# Autodesk Inventor assembly: Assembled_Olfactometer
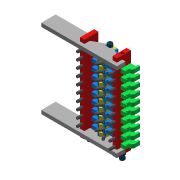
[picture p0: Inventor's stored thumbnail of the model, 180x180]
Saved by Autodesk Inventor 2016 (Build 200138000, 138)
## iProperties
Created: 2018-02-11
Part Number: Assembled_Olfactometer
Document SubType Name: Assembly
Designer: reinert
Author: reinert
## Documents named in this file (8)
- D:\PHD KUNER\Behaviour Setup\KunerOlfactometer_9Valves\Assembled_Olfactometer.iam
- D:\PHD KUNER\Behaviour Setup\KunerOlfactometer_9Valves\Olfactometer_Holder.ipt
- D:\PHD KUNER\Behaviour Setup\KunerOlfactometer_9Valves\OuterOlfactometerChannel.ipt
- D:\PHD KUNER\Behaviour Setup\KunerOlfactometer_9Valves\CentralManifold.ipt
- D:\PHD KUNER\Behaviour Setup\KunerOlfactometer_9Valves\Valve_Outside.ipt
- D:\PHD KUNER\Behaviour Setup\KunerOlfactometer_9Valves\Valve_Inside.ipt
- D:\PHD KUNER\Behaviour Setup\KunerOlfactometer_9Valves\KQ2S23_M5N_N.ipt
- D:\PHD KUNER\Behaviour Setup\KunerOlfactometer_9Valves\2027 CK-1_8-PK-4.ipt
## Components (89 placed, 7 different names)
1. Olfactometer_Holder:1 — Flush:1, Flush:2, Flush:3, Mate:1, Mate:3, Mate:4, Flush:5, Flush:6, Mate:5, Flush:9, Mate:6
2. Olfactometer_Holder:2 — Flush:1, Flush:2, Flush:3
3. OuterOlfactometerChannel:1 — Mate:1, Flush:9, Mate:6, Insert:1, Insert:2, Mate:8, Insert:11, Mate:14, Insert:16
4. OuterOlfactometerChannel:2 — Mate:3, Mate:4, Flush:5, Flush:8, Insert:3, Insert:4, Mate:7, Insert:9, Mate:13, Insert:15
5. CentralManifold:1 — Flush:6, Flush:8, Mate:5, Insert:5, Insert:6, Insert:7, Insert:8, Mate:9, Insert:10, Mate:10, Insert:12, Mate:11, Insert:13, Mate:12, Insert:14
6. 2027 CK-1_8-PK-4:1 — Mate:14, Insert:16
7. 2027 CK-1_8-PK-4:2 — Mate:12, Insert:14
8. 2027 CK-1_8-PK-4:3 — Mate:11, Insert:13
9. 2027 CK-1_8-PK-4:4 — Mate:13, Insert:15
10. Valve_Outside:1 — Insert:1, Insert:2
11. Valve_Outside:2
12. Valve_Outside:3
13. Valve_Outside:4
14. Valve_Outside:5
15. Valve_Outside:6
16. Valve_Outside:7
17. Valve_Outside:8
18. Valve_Outside:9
19. Valve_Outside:10
20. Valve_Outside:11 — Insert:3, Insert:4
21. Valve_Outside:12
22. Valve_Outside:13
23. Valve_Outside:14
24. Valve_Outside:15
25. Valve_Outside:16
26. Valve_Outside:17
27. Valve_Outside:18
28. Valve_Outside:19
29. Valve_Outside:20
30. Valve_Inside:1 — Insert:5, Insert:6
31. Valve_Inside:2
32. Valve_Inside:3
33. Valve_Inside:4
34. Valve_Inside:5
35. Valve_Inside:6
36. Valve_Inside:7
37. Valve_Inside:8
38. Valve_Inside:9
39. Valve_Inside:10
40. Valve_Inside:11 — Insert:7, Insert:8
41. Valve_Inside:12
42. Valve_Inside:13
43. Valve_Inside:14
44. Valve_Inside:15
45. Valve_Inside:16
46. Valve_Inside:17
47. Valve_Inside:18
48. Valve_Inside:19
49. Valve_Inside:20
50. KQ2S23_M5N_N:1 — Mate:7, Insert:9
51. KQ2S23_M5N_N:2
52. KQ2S23_M5N_N:3
53. KQ2S23_M5N_N:4
54. KQ2S23_M5N_N:5
55. KQ2S23_M5N_N:6
56. KQ2S23_M5N_N:7
57. KQ2S23_M5N_N:8
58. KQ2S23_M5N_N:9
59. KQ2S23_M5N_N:10
60. KQ2S23_M5N_N:11 — Mate:8, Insert:11
61. KQ2S23_M5N_N:14
62. KQ2S23_M5N_N:15
63. KQ2S23_M5N_N:16
64. KQ2S23_M5N_N:17
65. KQ2S23_M5N_N:18
66. KQ2S23_M5N_N:19
67. KQ2S23_M5N_N:20
68. KQ2S23_M5N_N:21
69. KQ2S23_M5N_N:22
70. KQ2S23_M5N_N:12 — Mate:9, Insert:10
71. KQ2S23_M5N_N:23
72. KQ2S23_M5N_N:24
73. KQ2S23_M5N_N:25
74. KQ2S23_M5N_N:26
75. KQ2S23_M5N_N:27
76. KQ2S23_M5N_N:28
77. KQ2S23_M5N_N:29
78. KQ2S23_M5N_N:30
79. KQ2S23_M5N_N:31
80. KQ2S23_M5N_N:13 — Mate:10, Insert:12
81. KQ2S23_M5N_N:32
82. KQ2S23_M5N_N:33
83. KQ2S23_M5N_N:34
84. KQ2S23_M5N_N:35
85. KQ2S23_M5N_N:36
86. KQ2S23_M5N_N:37
87. KQ2S23_M5N_N:38
88. KQ2S23_M5N_N:39
89. KQ2S23_M5N_N:40
## Component patterns: (10 elements, first: Valve_Outside:1), (10 elements, first: Valve_Outside:11), (10 elements, first: Valve_Inside:1), (10 elements, first: Valve_Inside:11), (10 elements, first: KQ2S23_M5N_N:1), (10 elements, first: KQ2S23_M5N_N:11), (10 elements, first: KQ2S23_M5N_N:12), (10 elements, first: KQ2S23_M5N_N:13)
## Relationships (36: Insert 16, Mate 13, Flush 7)
- Flush:1: Olfactometer_Holder:1 ↔ Olfactometer_Holder:2
- Flush:2: Olfactometer_Holder:1 ↔ Olfactometer_Holder:2
- Flush:3 (210 mm): Olfactometer_Holder:1 ↔ Olfactometer_Holder:2
- Mate:1: Olfactometer_Holder:1 ↔ OuterOlfactometerChannel:1
- Mate:3: Olfactometer_Holder:1 ↔ OuterOlfactometerChannel:2
- Mate:4: Olfactometer_Holder:1 ↔ OuterOlfactometerChannel:2
- Flush:5 (-10 mm): Olfactometer_Holder:1 ↔ OuterOlfactometerChannel:2
- Flush:6 (10 mm): Olfactometer_Holder:1 ↔ CentralManifold:1
- Flush:8 (7 mm): OuterOlfactometerChannel:2 ↔ CentralManifold:1
- Mate:5 (1.1 mm): Olfactometer_Holder:1 ↔ CentralManifold:1
- Flush:9 (-10 mm): Olfactometer_Holder:1 ↔ OuterOlfactometerChannel:1
- Mate:6: Olfactometer_Holder:1 ↔ OuterOlfactometerChannel:1
- Insert:1: OuterOlfactometerChannel:1 ↔ Valve_Outside:1
- Insert:2: OuterOlfactometerChannel:1 ↔ Valve_Outside:1
- Insert:3: OuterOlfactometerChannel:2 ↔ Valve_Outside:11
- Insert:4: OuterOlfactometerChannel:2 ↔ Valve_Outside:11
- Insert:5: CentralManifold:1 ↔ Valve_Inside:1
- Insert:6: CentralManifold:1 ↔ Valve_Inside:1
- Insert:7: CentralManifold:1 ↔ Valve_Inside:11
- Insert:8: CentralManifold:1 ↔ Valve_Inside:11
- Mate:7: OuterOlfactometerChannel:2 ↔ KQ2S23_M5N_N:1
- Insert:9: OuterOlfactometerChannel:2 ↔ KQ2S23_M5N_N:1
- Mate:8: OuterOlfactometerChannel:1 ↔ KQ2S23_M5N_N:11
- Mate:9: CentralManifold:1 ↔ KQ2S23_M5N_N:12
- Insert:10: CentralManifold:1 ↔ KQ2S23_M5N_N:12
- Insert:11: OuterOlfactometerChannel:1 ↔ KQ2S23_M5N_N:11
- Mate:10: CentralManifold:1 ↔ KQ2S23_M5N_N:13
- Insert:12: CentralManifold:1 ↔ KQ2S23_M5N_N:13
- Mate:11: CentralManifold:1 ↔ 2027 CK-1_8-PK-4:3
- Insert:13: CentralManifold:1 ↔ 2027 CK-1_8-PK-4:3
- Mate:12: CentralManifold:1 ↔ 2027 CK-1_8-PK-4:2
- Insert:14: CentralManifold:1 ↔ 2027 CK-1_8-PK-4:2
- Mate:13: OuterOlfactometerChannel:2 ↔ 2027 CK-1_8-PK-4:4
- Mate:14: OuterOlfactometerChannel:1 ↔ 2027 CK-1_8-PK-4:1
- Insert:15 (-10 mm): OuterOlfactometerChannel:2 ↔ 2027 CK-1_8-PK-4:4
- Insert:16: OuterOlfactometerChannel:1 ↔ 2027 CK-1_8-PK-4:1
